# Autodesk Inventor assembly: Rack and Pinion System
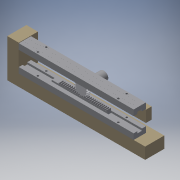
[picture p0: Inventor's stored thumbnail of the model, 180x180]
Saved by Autodesk Inventor 2016 (Build 200138000, 138)
## iProperties
Created: 2016-04-02
Part Number: Rack and Pinion System
Document SubType Name: Assembly
Designer: amycroft3
Author: amycroft3
## Documents named in this file (7)
- C:\Users\Ariana\Downloads\Capstone CAD\Capstone CAD\Rack and Pinion System.iam
- C:\Users\Ariana\Downloads\Capstone CAD\Capstone CAD\Rack and Pinion Gear.iam
- C:\Users\Ariana\Downloads\Capstone CAD\Capstone CAD\Rack and Pinion Wood Framing.ipt
- C:\Users\Ariana\Downloads\Capstone CAD\Capstone CAD\Rack Assembly.iam
- C:\Users\Ariana\Downloads\Capstone CAD\Capstone CAD\Rack and Pinion Frame Vertical.ipt
- C:\Users\Ariana\Downloads\Capstone CAD\Capstone CAD\Rack and Pinion Frame Back.ipt
- C:\Users\Ariana\Downloads\Capstone CAD\Capstone CAD\Motor + Attachment\Motor and Bracket for Rack and Pinion.iam
## Components (8 placed, 6 different names)
1. Rack and Pinion Wood Framing:1 — Flush:1, Mate:1, Flush:4, Mate:12, Mate:13, Flush:5, Flush:6, Flush:7, Flush:8
2. Rack Assembly:1 [sub-assembly] — Flush:2, Flush:3, Mate:16, Mate:20
3. Rack Assembly:2 [sub-assembly] — Flush:1, Mate:1, Flush:2, Flush:3, Flush:4, Mate:8, Mate:9
4. Rack and Pinion Gear:1 [sub-assembly] — Mate:8, Mate:9, Mate:16, Mate:18
5. Rack and Pinion Frame Vertical:1 — Mate:13, Flush:7, Flush:8
6. Rack and Pinion Frame Vertical:2 — Mate:12, Flush:5, Flush:6, Mate:14
7. Rack and Pinion Frame Back:1 — Mate:14, Mate:17, Angle:1, Mate:19, Mate:20
8. Motor and Bracket for Rack and Pinion:1 [sub-assembly] — Mate:17, Mate:18, Angle:1, Mate:19
## Relationships (20: Mate 11, Flush 8, Angle 1)
- Flush:1: Rack and Pinion Wood Framing:1 ↔ Rack Assembly:2
- Mate:1: Rack and Pinion Wood Framing:1 ↔ Rack Assembly:2
- Flush:2: Rack Assembly:1 ↔ Rack Assembly:2
- Flush:3: Rack Assembly:1 ↔ Rack Assembly:2
- Flush:4 (38.1 mm): Rack and Pinion Wood Framing:1 ↔ Rack Assembly:2
- Mate:8: Rack Assembly:2 ↔ Rack and Pinion Gear:1
- Mate:9: Rack Assembly:2 ↔ Rack and Pinion Gear:1
- Mate:12: Rack and Pinion Wood Framing:1 ↔ Rack and Pinion Frame Vertical:2
- Mate:13: Rack and Pinion Wood Framing:1 ↔ Rack and Pinion Frame Vertical:1
- Flush:5: Rack and Pinion Wood Framing:1 ↔ Rack and Pinion Frame Vertical:2
- Flush:6: Rack and Pinion Wood Framing:1 ↔ Rack and Pinion Frame Vertical:2
- Flush:7: Rack and Pinion Wood Framing:1 ↔ Rack and Pinion Frame Vertical:1
- Flush:8: Rack and Pinion Wood Framing:1 ↔ Rack and Pinion Frame Vertical:1
- Mate:14: Rack and Pinion Frame Vertical:2 ↔ Rack and Pinion Frame Back:1
- Mate:16: Rack Assembly:1 ↔ Rack and Pinion Gear:1
- Mate:17: Rack and Pinion Frame Back:1 ↔ Motor and Bracket for Rack and Pinion:1
- Mate:18: Rack and Pinion Gear:1 ↔ Motor and Bracket for Rack and Pinion:1
- Angle:1 (0 deg): Rack and Pinion Frame Back:1 ↔ Motor and Bracket for Rack and Pinion:1
- Mate:19 (190.5 mm): Rack and Pinion Frame Back:1 ↔ Motor and Bracket for Rack and Pinion:1
- Mate:20: Rack Assembly:1 ↔ Rack and Pinion Frame Back:1
